# Autodesk Inventor assembly: maxon motor
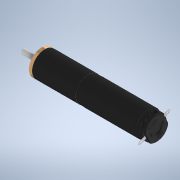
[picture p0: Inventor's stored thumbnail of the model, 180x180]
Saved by Autodesk Inventor 2020 (Build 240168000, 168)
## iProperties
Created: 2024-04-30
Part Number: maxon motor
Document SubType Name: Assembly
Designer: 4s
Author: 4s
## Documents named in this file (3)
- C:\Users\4s\Documents\Inventor models\Asterisk\robot_v2\maxon motor\maxon motor.iam
- C:\Users\4s\Documents\Inventor models\Asterisk\robot_v2\maxon motor\118710_RE16_GB_4_5W_SL_1WE.ipt
- C:\Users\4s\Documents\Inventor models\Asterisk\robot_v2\maxon gear\GP16A_5-Stufig-110325.ipt
## Components (2 placed, 2 different names)
1. 118710_RE16_GB_4_5W_SL_1WE:1 — Совмещение:1, Совмещение:2, Совмещение:3
2. GP16A_5-Stufig-110325:1 — Совмещение:1, Совмещение:2, Совмещение:3
## Relationships (3: Mate 3)
- Совмещение:1 [Mate]: 118710_RE16_GB_4_5W_SL_1WE:1 ↔ GP16A_5-Stufig-110325:1
- Совмещение:2 [Mate]: 118710_RE16_GB_4_5W_SL_1WE:1 ↔ GP16A_5-Stufig-110325:1
- Совмещение:3 [Mate]: 118710_RE16_GB_4_5W_SL_1WE:1 ↔ GP16A_5-Stufig-110325:1
